# Autodesk Inventor assembly: maze_prototip
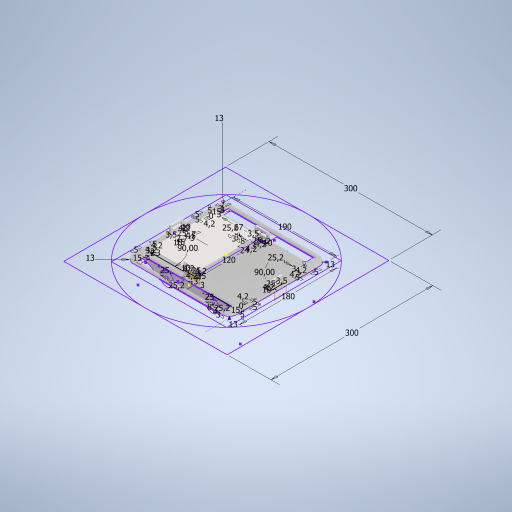
[picture p0: Inventor's stored thumbnail of the model, 512x512]
Saved by Autodesk Inventor 2023 (Build 270158000, 158)
## iProperties
Created: 2025-12-14
Part Number: maze_prototip
Document SubType Name: Assembly
Designer: garin
Author: garin
## Documents named in this file (6)
- C:\Users\garin\OneDrive\Документы\maze\maze_prototip.iam
- C:\Users\garin\OneDrive\Документы\maze\основа.ipt
- C:\Users\garin\OneDrive\Документы\maze\крепёж_для_мотора.ipt
- C:\Users\garin\OneDrive\Документы\maze\макетная плата.ipt
- C:\Users\garin\OneDrive\Документы\maze\крепление_RGB.ipt
- C:\Users\garin\OneDrive\Документы\maze\крепл_ЛД.ipt
## Components (9 placed, 5 different names)
1. основа:1 — С поворотом:1, С поворотом:2, Заподлицо:1, С поворотом:3, С поворотом:4, С поворотом:5, С поворотом:6, Жесткий:1, С поворотом:7, С поворотом:8, С поворотом:9
2. крепёж_для_мотора:1 — С поворотом:1
3. крепёж_для_мотора:2 — С поворотом:2
4. макетная плата:1 — Заподлицо:1
5. крепление_RGB:1 — С поворотом:3
6. крепл_ЛД:2 — С поворотом:6, С поворотом:8
7. крепл_ЛД:3 — С поворотом:5, С поворотом:9
8. крепл_ЛД:4 — С поворотом:4, С поворотом:7
9. крепл_ЛД:5 — Жесткий:1
## Relationships (11: RevoluteJoint 9, Flush 1, WeldJoint 1)
- С поворотом:1 [RevoluteJoint]: основа:1 ↔ крепёж_для_мотора:1
- С поворотом:2 [RevoluteJoint]: основа:1 ↔ крепёж_для_мотора:2
- Заподлицо:1 [Flush]: основа:1 ↔ макетная плата:1
- С поворотом:3 [RevoluteJoint]: основа:1 ↔ крепление_RGB:1
- С поворотом:4 [RevoluteJoint]: основа:1 ↔ крепл_ЛД:4
- С поворотом:5 [RevoluteJoint]: основа:1 ↔ крепл_ЛД:3
- С поворотом:6 [RevoluteJoint]: основа:1 ↔ крепл_ЛД:2
- Жесткий:1 [WeldJoint]: основа:1 ↔ крепл_ЛД:5
- С поворотом:7 [RevoluteJoint]: основа:1 ↔ крепл_ЛД:4
- С поворотом:8 [RevoluteJoint]: основа:1 ↔ крепл_ЛД:2
- С поворотом:9 [RevoluteJoint]: основа:1 ↔ крепл_ЛД:3
